# Autodesk Inventor assembly: Motor&MotorMount
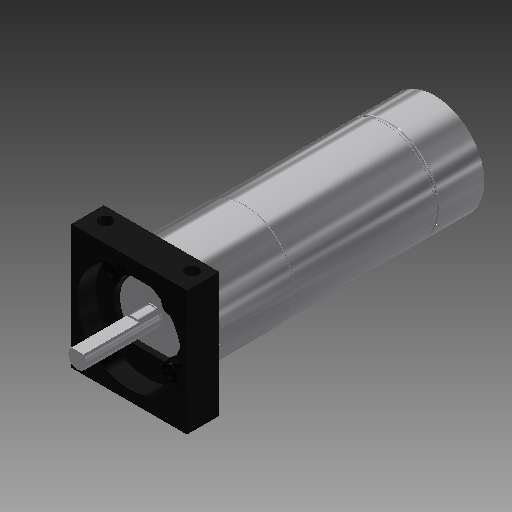
[picture p0: Inventor's stored thumbnail of the model, 512x512]
Saved by Autodesk Inventor 2017 (Build 210142000, 142)
## iProperties
Created: 2019-06-10
Part Number: Motor&MotorMount
Document SubType Name: Assembly
Designer: cresswnd
Author: cresswnd
## Documents named in this file (4)
- C:\Users\cresswnd\Documents\Robotics\Version 3\Concept_1\V2\Motor&MotorMount.iam
- C:\Users\cresswnd\Documents\Robotics\Version 3\Concept_1\V2\730RPM Motor Mockup.ipt
- C:\Users\cresswnd\Documents\Robotics\Version 3\Concept_1\V2\MotorMountv2.ipt
- C:\Users\cresswnd\Documents\Robotics\Version 3\Concept_1\V2\2x6mmScrew.ipt
## Components (6 placed, 3 different names)
1. 730RPM Motor Mockup:1 — Flush:1, Mate:1, Insert:1, Insert:2
2. MotorMountv2:1 — Flush:1, Mate:1, Insert:1, Insert:2, Insert:3, Insert:4, Insert:5, Insert:6
3. 2x6mmScrew:1 — Insert:3
4. 2x6mmScrew:2 — Insert:4
5. 2x6mmScrew:3 — Insert:5
6. 2x6mmScrew:4 — Insert:6
## Relationships (8: Insert 6, Flush 1, Mate 1)
- Flush:1: 730RPM Motor Mockup:1 ↔ MotorMountv2:1
- Mate:1: 730RPM Motor Mockup:1 ↔ MotorMountv2:1
- Insert:1: 730RPM Motor Mockup:1 ↔ MotorMountv2:1
- Insert:2: 730RPM Motor Mockup:1 ↔ MotorMountv2:1
- Insert:3: MotorMountv2:1 ↔ 2x6mmScrew:1
- Insert:4: MotorMountv2:1 ↔ 2x6mmScrew:2
- Insert:5: MotorMountv2:1 ↔ 2x6mmScrew:3
- Insert:6: MotorMountv2:1 ↔ 2x6mmScrew:4
